# Autodesk Inventor assembly: waist1
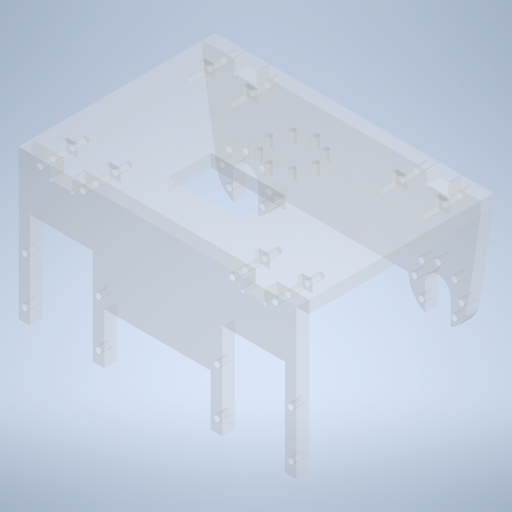
[picture p0: Inventor's stored thumbnail of the model, 512x512]
Saved by Autodesk Inventor 2024 (Build 280153000, 153)
## iProperties
Created: 2024-09-14
Part Number: waist1
Document SubType Name: Assembly
Designer: jmha0
Author: jmha0
## Documents named in this file (4)
- C:\Users\jmha0\OneDrive\바탕 화면\19th_intern_hjm_fight_robot\Lower_Body\waist\waist1.iam
- C:\Users\jmha0\OneDrive\바탕 화면\19th_intern_hjm_fight_robot\Lower_Body\waist\frame_waist_frames_linker1.ipt
- C:\Users\jmha0\OneDrive\바탕 화면\19th_intern_hjm_fight_robot\Lower_Body\waist\frame_pelvis_to_waist2.ipt
- C:\Users\jmha0\OneDrive\바탕 화면\19th_intern_hjm_fight_robot\Lower_Body\waist\frame_pelvis_to_waist1.ipt
## Components (3 placed, 3 different names)
1. frame_waist_frames_linker1:1 — 삽입:1, 삽입:2, 삽입:3, 삽입:4
2. frame_pelvis_to_waist2:1 — 삽입:1, 삽입:2
3. frame_pelvis_to_waist1:1 — 삽입:3, 삽입:4
## Relationships (4: Insert 4)
- 삽입:1 [Insert]: frame_waist_frames_linker1:1 ↔ frame_pelvis_to_waist2:1
- 삽입:2 [Insert]: frame_waist_frames_linker1:1 ↔ frame_pelvis_to_waist2:1
- 삽입:3 [Insert]: frame_waist_frames_linker1:1 ↔ frame_pelvis_to_waist1:1
- 삽입:4 [Insert]: frame_waist_frames_linker1:1 ↔ frame_pelvis_to_waist1:1
